# Autodesk Inventor assembly: Additional_Building_Version_2
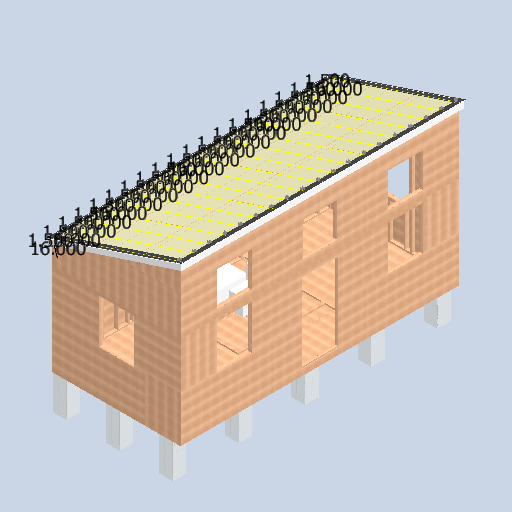
[picture p0: Inventor's stored thumbnail of the model, 512x512]
Saved by Autodesk Inventor 2025.1 (Build 291241020, 241B)
## iProperties
Created: 2024-10-03
Part Number: Additional_Building_Version_2
Document SubType Name: Assembly
Designer: Tom
Author: Tom
## Documents named in this file (31)
- C:\Users\Tom\Documents\Inventor\Mobility\Additional_Building\Additional_Building.iam
- C:\Users\Tom\Documents\Inventor\Mobility\Additional_Building\Grid_Of_Piers.iam
- C:\Users\Tom\Documents\Inventor\Mobility\Additional_Building\Floor_System.iam
- C:\Users\Tom\Documents\Inventor\Mobility\Additional_Building\Framing_For_First_Floor.iam
- C:\Users\Tom\Documents\Inventor\Mobility\Additional_Building\Framing_For_Roof.iam
- C:\Users\Tom\Documents\Inventor\Mobility\Additional_Building\Sheathing_For_Back.iam
- C:\Users\Tom\Documents\Inventor\Mobility\Additional_Building\Sheathing_For_Front.iam
- C:\Users\Tom\Documents\Inventor\Mobility\Additional_Building\Sheathing_For_Side.iam
- C:\Users\Tom\Documents\Inventor\Mobility\Additional_Building\Sheathing_For_Roof.iam
- C:\Users\Tom\Documents\Inventor\Mobility\Additional_Building\DensGlass.iam
- C:\Users\Tom\Documents\Inventor\Mobility\Additional_Building\Fascia_For_Back.ipt
- C:\Users\Tom\Documents\Inventor\Mobility\Additional_Building\Drip_Edge_For_Back_With_Length_97.504_Inches.ipt
- C:\Users\Tom\Documents\Inventor\Mobility\Additional_Building\Drip_Edge_For_Back_With_Length_48.752_Inches.ipt
- C:\Users\Tom\Documents\Inventor\Mobility\Additional_Building\Underlayment_Over_Back_Drip_Edge.ipt
- C:\Users\Tom\Documents\Inventor\Mobility\Additional_Building\Underlayment_Over_Underlayment_With_Width_36_Inches.ipt
- C:\Users\Tom\Documents\Inventor\Mobility\Additional_Building\Drip_Edge_For_Front_With_Length_48.919_Inches.ipt
- C:\Users\Tom\Documents\Inventor\Mobility\Additional_Building\Underlayment_Over_Underlayment_With_Width_9.865_Inches.ipt
- C:\Users\Tom\Documents\Inventor\Mobility\Additional_Building\Drip_Edge_For_Front_With_Length_97.837_Inches.ipt
- C:\Users\Tom\Documents\Inventor\Mobility\Additional_Building\Fascia_Vent_With_Length_13.75_Inches.ipt
- C:\Users\Tom\Documents\Inventor\Mobility\Additional_Building\Fascia_Vent_With_Length_14.5_Inches.ipt
- C:\Users\Tom\Documents\Inventor\Mobility\Additional_Building\Fascia_For_Front.ipt
- C:\Users\Tom\Documents\Inventor\Mobility\Additional_Building\Fascia_For_Side.ipt
- C:\Users\Tom\Documents\Inventor\Mobility\Additional_Building\Starter_Shingle_With_Dimensions_6.5_x_35_Inches.ipt
- C:\Users\Tom\Documents\Inventor\Mobility\Additional_Building\Starter_Shingle_With_Dimensions_6.5_x_38_Inches.ipt
- C:\Users\Tom\Documents\Inventor\Mobility\Additional_Building\Starter_Shingle_With_Dimensions_6.5_x_31.763_Inches.ipt
- C:\Users\Tom\Documents\Inventor\Mobility\Additional_Building\Starter_Shingle_With_Dimensions_6.5_x_28.25_Inches.ipt
- C:\Users\Tom\Documents\Inventor\Mobility\Additional_Building\Starter_Shingle_With_Dimensions_6.5_x_25.263_Inches.ipt
- C:\Users\Tom\Documents\Inventor\Mobility\Additional_Building\Starter_Shingle_With_Dimensions_6.5_x_38_Inches_With_Raise.ipt
- C:\Users\Tom\Documents\Inventor\Mobility\Additional_Building\Starter_Shingle_With_Dimensions_6.5_x_30.429_Inches.ipt
- C:\Users\Tom\Documents\Inventor\Mobility\Additional_Building\Drip_Edge_For_Side.ipt
- C:\Users\Tom\Documents\Inventor\Mobility\Additional_Building\Framing_For_Second_Floor.iam
## Components (76 placed, 30 different names)
1. Grid_Of_Piers:1 [sub-assembly] — Mate:57, Mate:58, Mate:59, Mate:74, Flush:50, Mate:75
2. Floor_System:1 [sub-assembly] — Mate:74, Flush:50, Mate:75, Flush:55, Mate:82, Mate:86, Flush:62, Flush:63, Flush:64
3. Framing_For_First_Floor:1 [sub-assembly] — Mate:3, Flush:5, Flush:6, Mate:4, Flush:8, Mate:5, Mate:86, Flush:62, Mate:87, Flush:65, Flush:66
4. Framing_For_Roof:1 [sub-assembly] — Mate:3, Flush:5, Flush:6, Flush:13, Flush:14, Mate:7, Mate:14, Mate:28, Mate:32, Mate:34, Mate:35, Flush:30, Mate:36, Mate:37, Flush:31, Mate:38
5. Sheathing_For_Back:1 [sub-assembly] — Mate:4, Flush:8, Mate:8, Flush:53, Flush:54, Flush:56, Flush:61, Flush:63
6. Sheathing_For_Front:1 [sub-assembly] — Mate:5, Flush:49, Flush:52, Flush:55, Flush:60
7. Sheathing_For_Roof:1 [sub-assembly] — Flush:13, Flush:14, Mate:7, Mate:11, Flush:21, Mate:15, Mate:27, Flush:34
8. Sheathing_For_Side:1 [sub-assembly] — Flush:16, Flush:49, Flush:52, Flush:53, Flush:56
9. DensGlass:1 [sub-assembly] — Mate:8, Flush:16, Flush:54, Flush:64
10. Underlayment_Over_Back_Drip_Edge:1 — Mate:19, Mate:20, Flush:24, Mate:21, Mate:22, Flush:25, Mate:76, Mate:84
11. Underlayment_Over_Underlayment_With_Width_36_Inches:1 — Mate:21, Mate:22, Flush:25, Mate:23, Mate:24, Flush:26
12. Underlayment_Over_Underlayment_With_Width_36_Inches:2 — Mate:23, Mate:24, Flush:26, Mate:25, Mate:26, Flush:27
13. Underlayment_Over_Underlayment_With_Width_36_Inches:3 — Mate:25, Mate:26, Flush:27, Mate:29, Mate:30, Flush:29
14. Underlayment_Over_Underlayment_With_Width_9.865_Inches:1 — Mate:29, Mate:30, Flush:29, Mate:31
15. Starter_Shingle_With_Dimensions_6.5_x_35_Inches:1 — Mate:48, Mate:50, Flush:36, Flush:37
16. Starter_Shingle_With_Dimensions_6.5_x_31.763_Inches:1 — Flush:38, Mate:67, Flush:44, Flush:58, Mate:80, Flush:59
17. Starter_Shingle_With_Dimensions_6.5_x_28.25_Inches:1 — Mate:61, Mate:64, Flush:42, Mate:73, Flush:47
18. Starter_Shingle_With_Dimensions_6.5_x_25.263_Inches:1 — Mate:65, Mate:66, Flush:43
19. Drip_Edge_For_Side:1 — Mate:76, Mate:77, Mate:78, Mate:79, Mate:81
20. Sheathing_For_Side:2 [sub-assembly] — Mate:82, Flush:60, Flush:61
21. Drip_Edge_For_Side:2 — Mate:83, Mate:84, Mate:85
22. Framing_For_Second_Floor:1 [sub-assembly] — Mate:87, Flush:65, Flush:66
23. Fascia_For_Back:1 — Mate:14, Flush:21, Flush:23, Mate:16, Mate:40, Flush:35
24. Fascia_For_Back:2 — Mate:17
25. Fascia_For_Back:3
26. Drip_Edge_For_Back_With_Length_97.504_Inches:1 — Mate:11, Mate:17, Mate:18
27. Drip_Edge_For_Back_With_Length_97.504_Inches:2
28. Drip_Edge_For_Back_With_Length_48.752_Inches:1 — Mate:15, Flush:23, Mate:16, Mate:18, Mate:19, Mate:20, Flush:24
29. Drip_Edge_For_Back_With_Length_48.752_Inches:2 — Mate:48
30. Drip_Edge_For_Front_With_Length_97.837_Inches:1 — Mate:31, Mate:32, Mate:33
31. Drip_Edge_For_Front_With_Length_97.837_Inches:2 — Mate:63
32. Drip_Edge_For_Front_With_Length_48.919_Inches:1 — Mate:27, Mate:28, Mate:33, Mate:39, Mate:65, Mate:71, Mate:72, Mate:77
33. Drip_Edge_For_Front_With_Length_48.919_Inches:2 — Mate:61, Mate:83
34. Fascia_Vent_With_Length_14.5_Inches:1 — Mate:36, Mate:37, Flush:31
35. Fascia_Vent_With_Length_14.5_Inches:2
36. Fascia_Vent_With_Length_14.5_Inches:3
37. Fascia_Vent_With_Length_14.5_Inches:4
38. Fascia_Vent_With_Length_14.5_Inches:5
39. Fascia_Vent_With_Length_14.5_Inches:6
40. Fascia_Vent_With_Length_14.5_Inches:7
41. Fascia_Vent_With_Length_14.5_Inches:8
42. Fascia_Vent_With_Length_14.5_Inches:9
43. Fascia_Vent_With_Length_14.5_Inches:10
44. Fascia_Vent_With_Length_14.5_Inches:11
45. Fascia_Vent_With_Length_14.5_Inches:12
46. Fascia_Vent_With_Length_14.5_Inches:13
47. Fascia_Vent_With_Length_14.5_Inches:14
48. Fascia_Vent_With_Length_14.5_Inches:15
49. Fascia_Vent_With_Length_14.5_Inches:16
50. Fascia_Vent_With_Length_13.75_Inches:1 — Mate:34, Mate:35, Flush:30
51. Fascia_Vent_With_Length_13.75_Inches:2
52. Fascia_For_Front:1 — Mate:38, Mate:39
53. Fascia_For_Front:2
54. Fascia_For_Front:3
55. Fascia_For_Side:1 — Mate:40, Flush:34, Flush:35, Mate:78
56. Fascia_For_Side:2 — Mate:85
57. Starter_Shingle_With_Dimensions_6.5_x_38_Inches:1 — Mate:50, Flush:36, Flush:37
58. Starter_Shingle_With_Dimensions_6.5_x_38_Inches:2
59. Starter_Shingle_With_Dimensions_6.5_x_38_Inches:3
60. Starter_Shingle_With_Dimensions_6.5_x_38_Inches:4
61. Starter_Shingle_With_Dimensions_6.5_x_38_Inches:5
62. Starter_Shingle_With_Dimensions_6.5_x_38_Inches:6 — Flush:38, Flush:58
63. Starter_Shingle_With_Dimensions_6.5_x_38_Inches:13 — Mate:63, Mate:64, Flush:42
64. Starter_Shingle_With_Dimensions_6.5_x_38_Inches:14
65. Starter_Shingle_With_Dimensions_6.5_x_38_Inches:15
66. Starter_Shingle_With_Dimensions_6.5_x_38_Inches:16
67. Starter_Shingle_With_Dimensions_6.5_x_38_Inches:17
68. Starter_Shingle_With_Dimensions_6.5_x_38_Inches:18 — Mate:66, Flush:43
69. Starter_Shingle_With_Dimensions_6.5_x_38_Inches_With_Raise:1 — Mate:67, Flush:44, Mate:70, Flush:46, Mate:79, Mate:80, Mate:81, Flush:59
70. Starter_Shingle_With_Dimensions_6.5_x_30.429_Inches:1 — Mate:71, Mate:72, Flush:45, Flush:57
71. Starter_Shingle_With_Dimensions_6.5_x_38_Inches_With_Raise:2
72. Starter_Shingle_With_Dimensions_6.5_x_30.429_Inches:2 — Mate:73, Flush:47
73. Starter_Shingle_With_Dimensions_6.5_x_38_Inches:19 — Mate:70, Flush:46, Flush:57
74. Starter_Shingle_With_Dimensions_6.5_x_38_Inches:20 — Flush:45
75. Starter_Shingle_With_Dimensions_6.5_x_38_Inches:21
76. Starter_Shingle_With_Dimensions_6.5_x_38_Inches:22
## Component patterns: (3 elements, first: Fascia_For_Back:1), (2 elements, first: Drip_Edge_For_Back_With_Length_97.504_Inches:1), (2 elements, first: Drip_Edge_For_Back_With_Length_48.752_Inches:1), (2 elements, first: Drip_Edge_For_Front_With_Length_97.837_Inches:1), (2 elements, first: Drip_Edge_For_Front_With_Length_48.919_Inches:1), (16 elements, first: Fascia_Vent_With_Length_14.5_Inches:1), (2 elements, first: Fascia_Vent_With_Length_13.75_Inches:1), (3 elements, first: Fascia_For_Front:1), (2 elements, first: Fascia_For_Side:1), (6 elements, first: Starter_Shingle_With_Dimensions_6.5_x_38_Inches:1), (6 elements, first: Starter_Shingle_With_Dimensions_6.5_x_38_Inches:13), (2 elements, first: Starter_Shingle_With_Dimensions_6.5_x_38_Inches_With_Raise:1 + Starter_Shingle_With_Dimensions_6.5_x_30.429_Inches:1), (2 elements, first: Starter_Shingle_With_Dimensions_6.5_x_38_Inches:19), Component Pattern 17:2 (2 elements)
## Relationships (105: Mate 62, Flush 43)
- Mate:3 (1079.5 mm): Framing_For_First_Floor:1 ↔ Framing_For_Roof:1
- Flush:5: Framing_For_First_Floor:1 ↔ Framing_For_Roof:1
- Flush:6: Framing_For_First_Floor:1 ↔ Framing_For_Roof:1
- Mate:4: Framing_For_First_Floor:1 ↔ Sheathing_For_Back:1
- Flush:8: Framing_For_First_Floor:1 ↔ Sheathing_For_Back:1
- Mate:5: Framing_For_First_Floor:1 ↔ Sheathing_For_Front:1
- Flush:13: Framing_For_Roof:1 ↔ Sheathing_For_Roof:1
- Flush:14: Framing_For_Roof:1 ↔ Sheathing_For_Roof:1
- Mate:7: Framing_For_Roof:1 ↔ Sheathing_For_Roof:1
- Mate:8: Sheathing_For_Back:1 ↔ DensGlass:1
- Flush:16: Sheathing_For_Side:1 ↔ DensGlass:1
- Mate:11: Sheathing_For_Roof:1 ↔ Drip_Edge_For_Back_With_Length_97.504_Inches:1
- Mate:14: Framing_For_Roof:1 ↔ Fascia_For_Back:1
- Flush:21: Sheathing_For_Roof:1 ↔ Fascia_For_Back:1
- Mate:15: Sheathing_For_Roof:1 ↔ Drip_Edge_For_Back_With_Length_48.752_Inches:1
- Flush:23: Fascia_For_Back:1 ↔ Drip_Edge_For_Back_With_Length_48.752_Inches:1
- Mate:16: Fascia_For_Back:1 ↔ Drip_Edge_For_Back_With_Length_48.752_Inches:1
- Mate:17: Fascia_For_Back:2 ↔ Drip_Edge_For_Back_With_Length_97.504_Inches:1
- Mate:18: Drip_Edge_For_Back_With_Length_97.504_Inches:1 ↔ Drip_Edge_For_Back_With_Length_48.752_Inches:1
- Mate:19: Underlayment_Over_Back_Drip_Edge:1 ↔ Drip_Edge_For_Back_With_Length_48.752_Inches:1
- Mate:20: Underlayment_Over_Back_Drip_Edge:1 ↔ Drip_Edge_For_Back_With_Length_48.752_Inches:1
- Flush:24: Underlayment_Over_Back_Drip_Edge:1 ↔ Drip_Edge_For_Back_With_Length_48.752_Inches:1
- Mate:21: Underlayment_Over_Back_Drip_Edge:1 ↔ Underlayment_Over_Underlayment_With_Width_36_Inches:1
- Mate:22: Underlayment_Over_Back_Drip_Edge:1 ↔ Underlayment_Over_Underlayment_With_Width_36_Inches:1
- Flush:25: Underlayment_Over_Back_Drip_Edge:1 ↔ Underlayment_Over_Underlayment_With_Width_36_Inches:1
- Mate:23: Underlayment_Over_Underlayment_With_Width_36_Inches:1 ↔ Underlayment_Over_Underlayment_With_Width_36_Inches:2
- Mate:24: Underlayment_Over_Underlayment_With_Width_36_Inches:1 ↔ Underlayment_Over_Underlayment_With_Width_36_Inches:2
- Flush:26: Underlayment_Over_Underlayment_With_Width_36_Inches:1 ↔ Underlayment_Over_Underlayment_With_Width_36_Inches:2
- Mate:25: Underlayment_Over_Underlayment_With_Width_36_Inches:2 ↔ Underlayment_Over_Underlayment_With_Width_36_Inches:3
- Mate:26: Underlayment_Over_Underlayment_With_Width_36_Inches:2 ↔ Underlayment_Over_Underlayment_With_Width_36_Inches:3
- Flush:27: Underlayment_Over_Underlayment_With_Width_36_Inches:2 ↔ Underlayment_Over_Underlayment_With_Width_36_Inches:3
- Mate:27 (9.525 mm): Sheathing_For_Roof:1 ↔ Drip_Edge_For_Front_With_Length_48.919_Inches:1
- Mate:28 (25.4 mm): Framing_For_Roof:1 ↔ Drip_Edge_For_Front_With_Length_48.919_Inches:1
- Mate:29: Underlayment_Over_Underlayment_With_Width_36_Inches:3 ↔ Underlayment_Over_Underlayment_With_Width_9.865_Inches:1
- Mate:30: Underlayment_Over_Underlayment_With_Width_36_Inches:3 ↔ Underlayment_Over_Underlayment_With_Width_9.865_Inches:1
- Flush:29: Underlayment_Over_Underlayment_With_Width_36_Inches:3 ↔ Underlayment_Over_Underlayment_With_Width_9.865_Inches:1
- Mate:31 (6.35 mm): Underlayment_Over_Underlayment_With_Width_9.865_Inches:1 ↔ Drip_Edge_For_Front_With_Length_97.837_Inches:1
- Mate:32 (25.4 mm): Framing_For_Roof:1 ↔ Drip_Edge_For_Front_With_Length_97.837_Inches:1
- Mate:33: Drip_Edge_For_Front_With_Length_97.837_Inches:1 ↔ Drip_Edge_For_Front_With_Length_48.919_Inches:1
- Mate:34: Framing_For_Roof:1 ↔ Fascia_Vent_With_Length_13.75_Inches:1
- Mate:35: Framing_For_Roof:1 ↔ Fascia_Vent_With_Length_13.75_Inches:1
- Flush:30: Framing_For_Roof:1 ↔ Fascia_Vent_With_Length_13.75_Inches:1
- Mate:36: Framing_For_Roof:1 ↔ Fascia_Vent_With_Length_14.5_Inches:1
- Mate:37: Framing_For_Roof:1 ↔ Fascia_Vent_With_Length_14.5_Inches:1
- Flush:31: Framing_For_Roof:1 ↔ Fascia_Vent_With_Length_14.5_Inches:1
- Mate:38: Framing_For_Roof:1 ↔ Fascia_For_Front:1
- Mate:39 (3.175 mm): Drip_Edge_For_Front_With_Length_48.919_Inches:1 ↔ Fascia_For_Front:1
- Mate:40: Fascia_For_Back:1 ↔ Fascia_For_Side:1
- Flush:34: Sheathing_For_Roof:1 ↔ Fascia_For_Side:1
- Flush:35: Fascia_For_Back:1 ↔ Fascia_For_Side:1
- Mate:48 (-9.525 mm): Starter_Shingle_With_Dimensions_6.5_x_35_Inches:1 ↔ Drip_Edge_For_Back_With_Length_48.752_Inches:2
- Mate:50: Starter_Shingle_With_Dimensions_6.5_x_35_Inches:1 ↔ Starter_Shingle_With_Dimensions_6.5_x_38_Inches:1
- Flush:36: Starter_Shingle_With_Dimensions_6.5_x_35_Inches:1 ↔ Starter_Shingle_With_Dimensions_6.5_x_38_Inches:1
- Flush:37: Starter_Shingle_With_Dimensions_6.5_x_35_Inches:1 ↔ Starter_Shingle_With_Dimensions_6.5_x_38_Inches:1
- Flush:38: Starter_Shingle_With_Dimensions_6.5_x_31.763_Inches:1 ↔ Starter_Shingle_With_Dimensions_6.5_x_38_Inches:6
- Mate:57: Grid_Of_Piers:1
- Mate:58: Grid_Of_Piers:1
- Mate:59: Grid_Of_Piers:1
- Mate:61: Starter_Shingle_With_Dimensions_6.5_x_28.25_Inches:1 ↔ Drip_Edge_For_Front_With_Length_48.919_Inches:2
- Mate:63: Drip_Edge_For_Front_With_Length_97.837_Inches:2 ↔ Starter_Shingle_With_Dimensions_6.5_x_38_Inches:13
- Mate:64: Starter_Shingle_With_Dimensions_6.5_x_28.25_Inches:1 ↔ Starter_Shingle_With_Dimensions_6.5_x_38_Inches:13
- Flush:42: Starter_Shingle_With_Dimensions_6.5_x_28.25_Inches:1 ↔ Starter_Shingle_With_Dimensions_6.5_x_38_Inches:13
- Mate:65: Starter_Shingle_With_Dimensions_6.5_x_25.263_Inches:1 ↔ Drip_Edge_For_Front_With_Length_48.919_Inches:1
- Mate:66: Starter_Shingle_With_Dimensions_6.5_x_25.263_Inches:1 ↔ Starter_Shingle_With_Dimensions_6.5_x_38_Inches:18
- Flush:43: Starter_Shingle_With_Dimensions_6.5_x_25.263_Inches:1 ↔ Starter_Shingle_With_Dimensions_6.5_x_38_Inches:18
- Mate:67: Starter_Shingle_With_Dimensions_6.5_x_31.763_Inches:1 ↔ Starter_Shingle_With_Dimensions_6.5_x_38_Inches_With_Raise:1
- Flush:44: Starter_Shingle_With_Dimensions_6.5_x_31.763_Inches:1 ↔ Starter_Shingle_With_Dimensions_6.5_x_38_Inches_With_Raise:1
- Mate:70: Starter_Shingle_With_Dimensions_6.5_x_38_Inches_With_Raise:1 ↔ Starter_Shingle_With_Dimensions_6.5_x_38_Inches:19
- Mate:71: Drip_Edge_For_Front_With_Length_48.919_Inches:1 ↔ Starter_Shingle_With_Dimensions_6.5_x_30.429_Inches:1
- Mate:72: Drip_Edge_For_Front_With_Length_48.919_Inches:1 ↔ Starter_Shingle_With_Dimensions_6.5_x_30.429_Inches:1
- Flush:45: Starter_Shingle_With_Dimensions_6.5_x_30.429_Inches:1 ↔ Starter_Shingle_With_Dimensions_6.5_x_38_Inches:20
- Flush:46: Starter_Shingle_With_Dimensions_6.5_x_38_Inches_With_Raise:1 ↔ Starter_Shingle_With_Dimensions_6.5_x_38_Inches:19
- Mate:73: Starter_Shingle_With_Dimensions_6.5_x_28.25_Inches:1 ↔ Starter_Shingle_With_Dimensions_6.5_x_30.429_Inches:2
- Flush:47: Starter_Shingle_With_Dimensions_6.5_x_28.25_Inches:1 ↔ Starter_Shingle_With_Dimensions_6.5_x_30.429_Inches:2
- Flush:49: Sheathing_For_Front:1 ↔ Sheathing_For_Side:1
- Mate:74: Grid_Of_Piers:1 ↔ Floor_System:1
- Flush:50: Grid_Of_Piers:1 ↔ Floor_System:1
- Mate:75: Grid_Of_Piers:1 ↔ Floor_System:1
- Flush:52: Sheathing_For_Front:1 ↔ Sheathing_For_Side:1
- Flush:53: Sheathing_For_Back:1 ↔ Sheathing_For_Side:1
- Flush:54: Sheathing_For_Back:1 ↔ DensGlass:1
- Flush:55: Floor_System:1 ↔ Sheathing_For_Front:1
- Flush:56: Sheathing_For_Back:1 ↔ Sheathing_For_Side:1
- Flush:57: Starter_Shingle_With_Dimensions_6.5_x_30.429_Inches:1 ↔ Starter_Shingle_With_Dimensions_6.5_x_38_Inches:19
- Mate:76: Underlayment_Over_Back_Drip_Edge:1 ↔ Drip_Edge_For_Side:1
- Mate:77: Drip_Edge_For_Side:1 ↔ Drip_Edge_For_Front_With_Length_48.919_Inches:1
- Mate:78: Drip_Edge_For_Side:1 ↔ Fascia_For_Side:1
- Mate:79: Drip_Edge_For_Side:1 ↔ Starter_Shingle_With_Dimensions_6.5_x_38_Inches_With_Raise:1
- Flush:58: Starter_Shingle_With_Dimensions_6.5_x_31.763_Inches:1 ↔ Starter_Shingle_With_Dimensions_6.5_x_38_Inches:6
- Mate:80: Starter_Shingle_With_Dimensions_6.5_x_31.763_Inches:1 ↔ Starter_Shingle_With_Dimensions_6.5_x_38_Inches_With_Raise:1
- Mate:81 (-12.7 mm): Drip_Edge_For_Side:1 ↔ Starter_Shingle_With_Dimensions_6.5_x_38_Inches_With_Raise:1
- Flush:59: Starter_Shingle_With_Dimensions_6.5_x_31.763_Inches:1 ↔ Starter_Shingle_With_Dimensions_6.5_x_38_Inches_With_Raise:1
- Mate:82: Floor_System:1 ↔ Sheathing_For_Side:2
- Flush:60: Sheathing_For_Front:1 ↔ Sheathing_For_Side:2
- Flush:61: Sheathing_For_Back:1 ↔ Sheathing_For_Side:2
- Mate:83: Drip_Edge_For_Side:2 ↔ Drip_Edge_For_Front_With_Length_48.919_Inches:2
- Mate:84: Underlayment_Over_Back_Drip_Edge:1 ↔ Drip_Edge_For_Side:2
- Mate:85: Drip_Edge_For_Side:2 ↔ Fascia_For_Side:2
- Mate:86: Floor_System:1 ↔ Framing_For_First_Floor:1
- Flush:62: Floor_System:1 ↔ Framing_For_First_Floor:1
- Flush:63: Floor_System:1 ↔ Sheathing_For_Back:1
- Flush:64 (-12.7 mm): Floor_System:1 ↔ DensGlass:1
- Mate:87: Framing_For_First_Floor:1 ↔ Framing_For_Second_Floor:1
- Flush:65: Framing_For_First_Floor:1 ↔ Framing_For_Second_Floor:1
- Flush:66: Framing_For_First_Floor:1 ↔ Framing_For_Second_Floor:1
